# Autodesk Inventor assembly: zlozenie_ramka
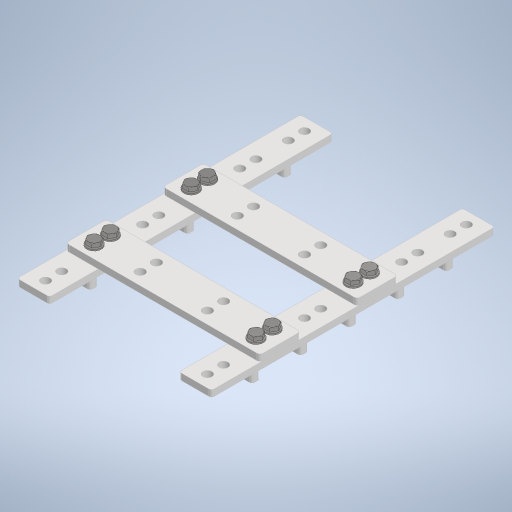
[picture p0: Inventor's stored thumbnail of the model, 512x512]
Saved by Autodesk Inventor 2024.2 (Build 282272000, 272)
## iProperties
Created: 2024-01-20
Part Number: zlozenie_ramka
Document SubType Name: Assembly
Designer: Konrad
Author: Konrad
## Documents named in this file (6)
- D:\Inventor\magisterka\prototyp_2\zlozenie_ramka.iam
- D:\Inventor\magisterka\prototyp_2\belka_poprzeg.ipt
- D:\Inventor\magisterka\prototyp_2\belka_wzdluz.ipt
- C:\Users\Konrad\Documents\Inventor\Content Center Files\R2024\pl-PL\DIN 125-1  A\DIN 125 - A 4,3.ipt
- C:\Users\Konrad\Documents\Inventor\Content Center Files\R2024\pl-PL\DIN EN 24 017\ISO 4017 - M4 x 16DIN EN.ipt
- C:\Users\Konrad\Documents\Inventor\Content Center Files\R2024\pl-PL\DIN 934\DIN 934 - M4 x 0,7.ipt
## Components (28 placed, 5 different names)
1. belka_poprzeg:1 — Zestawiające:1, Zestawiające:2, Równoległe:1, Równoległe:2, Zestawiające:4, Zestawiające:25, Zestawiające:27, Zestawiające:29, Zestawiające:31, Zestawiające:33, Zestawiające:35, Zestawiające:37, Zestawiające:39, Zestawiające:40, Zestawiające:41
2. belka_wzdluz:1 — Zestawiające:2, Równoległe:1, Zestawiające:4, Zestawiające:6, Zestawiające:16, Zestawiające:18, Zestawiające:20, Zestawiające:22, Zestawiające:32, Zestawiające:34, Zestawiające:36, Zestawiające:38
3. belka_poprzeg:2 — Zestawiające:3, Zestawiające:6, Zestawiające:42
4. belka_wzdluz:2 — Zestawiające:1, Równoległe:2, Zestawiające:3, Zestawiające:8, Zestawiające:9, Zestawiające:10, Zestawiające:11, Zestawiające:12, Zestawiające:13, Zestawiające:14, Zestawiające:15, Zestawiające:17, Zestawiające:19, Zestawiające:21, Zestawiające:23, Zestawiające:24, Zestawiające:26, Zestawiające:28, Zestawiające:30, Zestawiające:41, Zestawiające:42
5. DIN 125-1 A A 4,3:1 — Zestawiające:8, Zestawiające:9, Wstawiające:1
6. DIN EN 24017 M4 x 16:1 — Wstawiające:1
7. DIN 934 - zastąpiona przez DIN EN 24032/28673/28674 M4:1 — Zestawiające:24, Zestawiające:25
8. DIN 125-1 A A 4,3:2 — Zestawiające:10, Zestawiające:11, Wstawiające:2
9. DIN 125-1 A A 4,3:3 — Zestawiające:12, Zestawiające:13, Wstawiające:3
10. DIN 125-1 A A 4,3:4 — Zestawiające:14, Zestawiające:15, Wstawiające:4
11. DIN 125-1 A A 4,3:5 — Zestawiające:16, Zestawiające:17, Wstawiające:5
12. DIN 125-1 A A 4,3:6 — Zestawiające:18, Zestawiające:19, Wstawiające:6
13. DIN 125-1 A A 4,3:7 — Zestawiające:20, Zestawiające:21, Wstawiające:7
14. DIN 125-1 A A 4,3:8 — Zestawiające:22, Zestawiające:23, Wstawiające:8
15. DIN EN 24017 M4 x 16:2 — Wstawiające:2
16. DIN EN 24017 M4 x 16:3 — Wstawiające:3
17. DIN EN 24017 M4 x 16:4 — Wstawiające:4
18. DIN EN 24017 M4 x 16:5 — Wstawiające:5
19. DIN EN 24017 M4 x 16:6 — Wstawiające:6
20. DIN EN 24017 M4 x 16:7 — Wstawiające:7
21. DIN EN 24017 M4 x 16:8 — Wstawiające:8
22. DIN 934 - zastąpiona przez DIN EN 24032/28673/28674 M4:2 — Zestawiające:26, Zestawiające:27
23. DIN 934 - zastąpiona przez DIN EN 24032/28673/28674 M4:3 — Zestawiające:28, Zestawiające:29
24. DIN 934 - zastąpiona przez DIN EN 24032/28673/28674 M4:4 — Zestawiające:30, Zestawiające:31
25. DIN 934 - zastąpiona przez DIN EN 24032/28673/28674 M4:5 — Zestawiające:32, Zestawiające:33
26. DIN 934 - zastąpiona przez DIN EN 24032/28673/28674 M4:6 — Zestawiające:34, Zestawiające:35
27. DIN 934 - zastąpiona przez DIN EN 24032/28673/28674 M4:7 — Zestawiające:36, Zestawiające:37
28. DIN 934 - zastąpiona przez DIN EN 24032/28673/28674 M4:8 — Zestawiające:38, Zestawiające:39
## Relationships (50: Mate 40, Insert 8, Flush 2)
- Zestawiające:1 [Mate]: belka_poprzeg:1 ↔ belka_wzdluz:2
- Zestawiające:2 [Mate]: belka_poprzeg:1 ↔ belka_wzdluz:1
- Równoległe:1 [Flush]: belka_poprzeg:1 ↔ belka_wzdluz:1
- Równoległe:2 [Flush]: belka_poprzeg:1 ↔ belka_wzdluz:2
- Zestawiające:3 [Mate]: belka_poprzeg:2 ↔ belka_wzdluz:2
- Zestawiające:4 [Mate]: belka_poprzeg:1 ↔ belka_wzdluz:1
- Zestawiające:6 [Mate]: belka_wzdluz:1 ↔ belka_poprzeg:2
- Zestawiające:8 [Mate]: belka_wzdluz:2 ↔ DIN 125-1 A A 4,3:1
- Zestawiające:9 [Mate]: belka_wzdluz:2 ↔ DIN 125-1 A A 4,3:1
- Zestawiające:10 [Mate]: belka_wzdluz:2 ↔ DIN 125-1 A A 4,3:2
- Zestawiające:11 [Mate]: belka_wzdluz:2 ↔ DIN 125-1 A A 4,3:2
- Zestawiające:12 [Mate]: belka_wzdluz:2 ↔ DIN 125-1 A A 4,3:3
- Zestawiające:13 [Mate]: belka_wzdluz:2 ↔ DIN 125-1 A A 4,3:3
- Zestawiające:14 [Mate]: belka_wzdluz:2 ↔ DIN 125-1 A A 4,3:4
- Zestawiające:15 [Mate]: belka_wzdluz:2 ↔ DIN 125-1 A A 4,3:4
- Zestawiające:16 [Mate]: belka_wzdluz:1 ↔ DIN 125-1 A A 4,3:5
- Zestawiające:17 [Mate]: belka_wzdluz:2 ↔ DIN 125-1 A A 4,3:5
- Zestawiające:18 [Mate]: belka_wzdluz:1 ↔ DIN 125-1 A A 4,3:6
- Zestawiające:19 [Mate]: belka_wzdluz:2 ↔ DIN 125-1 A A 4,3:6
- Zestawiające:20 [Mate]: belka_wzdluz:1 ↔ DIN 125-1 A A 4,3:7
- Zestawiające:21 [Mate]: belka_wzdluz:2 ↔ DIN 125-1 A A 4,3:7
- Zestawiające:22 [Mate]: belka_wzdluz:1 ↔ DIN 125-1 A A 4,3:8
- Zestawiające:23 [Mate]: belka_wzdluz:2 ↔ DIN 125-1 A A 4,3:8
- Wstawiające:1 [Insert]: DIN 125-1 A A 4,3:1 ↔ DIN EN 24017 M4 x 16:1
- Wstawiające:2 [Insert]: DIN 125-1 A A 4,3:2 ↔ DIN EN 24017 M4 x 16:2
- Wstawiające:3 [Insert]: DIN 125-1 A A 4,3:3 ↔ DIN EN 24017 M4 x 16:3
- Wstawiające:4 [Insert]: DIN 125-1 A A 4,3:4 ↔ DIN EN 24017 M4 x 16:4
- Wstawiające:5 [Insert]: DIN 125-1 A A 4,3:5 ↔ DIN EN 24017 M4 x 16:5
- Wstawiające:6 [Insert]: DIN 125-1 A A 4,3:6 ↔ DIN EN 24017 M4 x 16:6
- Wstawiające:7 [Insert]: DIN 125-1 A A 4,3:7 ↔ DIN EN 24017 M4 x 16:7
- Wstawiające:8 [Insert]: DIN 125-1 A A 4,3:8 ↔ DIN EN 24017 M4 x 16:8
- Zestawiające:24 [Mate]: belka_wzdluz:2 ↔ DIN 934 - zastąpiona przez DIN EN 24032/28673/28674 M4:1
- Zestawiające:25 [Mate]: belka_poprzeg:1 ↔ DIN 934 - zastąpiona przez DIN EN 24032/28673/28674 M4:1
- Zestawiające:26 [Mate]: belka_wzdluz:2 ↔ DIN 934 - zastąpiona przez DIN EN 24032/28673/28674 M4:2
- Zestawiające:27 [Mate]: belka_poprzeg:1 ↔ DIN 934 - zastąpiona przez DIN EN 24032/28673/28674 M4:2
- Zestawiające:28 [Mate]: belka_wzdluz:2 ↔ DIN 934 - zastąpiona przez DIN EN 24032/28673/28674 M4:3
- Zestawiające:29 [Mate]: belka_poprzeg:1 ↔ DIN 934 - zastąpiona przez DIN EN 24032/28673/28674 M4:3
- Zestawiające:30 [Mate]: belka_wzdluz:2 ↔ DIN 934 - zastąpiona przez DIN EN 24032/28673/28674 M4:4
- Zestawiające:31 [Mate]: belka_poprzeg:1 ↔ DIN 934 - zastąpiona przez DIN EN 24032/28673/28674 M4:4
- Zestawiające:32 [Mate]: belka_wzdluz:1 ↔ DIN 934 - zastąpiona przez DIN EN 24032/28673/28674 M4:5
- Zestawiające:33 [Mate]: belka_poprzeg:1 ↔ DIN 934 - zastąpiona przez DIN EN 24032/28673/28674 M4:5
- Zestawiające:34 [Mate]: belka_wzdluz:1 ↔ DIN 934 - zastąpiona przez DIN EN 24032/28673/28674 M4:6
- Zestawiające:35 [Mate]: belka_poprzeg:1 ↔ DIN 934 - zastąpiona przez DIN EN 24032/28673/28674 M4:6
- Zestawiające:36 [Mate]: belka_wzdluz:1 ↔ DIN 934 - zastąpiona przez DIN EN 24032/28673/28674 M4:7
- Zestawiające:37 [Mate]: belka_poprzeg:1 ↔ DIN 934 - zastąpiona przez DIN EN 24032/28673/28674 M4:7
- Zestawiające:38 [Mate]: belka_wzdluz:1 ↔ DIN 934 - zastąpiona przez DIN EN 24032/28673/28674 M4:8
- Zestawiające:39 [Mate]: belka_poprzeg:1 ↔ DIN 934 - zastąpiona przez DIN EN 24032/28673/28674 M4:8
- Zestawiające:40 [Mate]: belka_poprzeg:1
- Zestawiające:41 [Mate]: belka_poprzeg:1 ↔ belka_wzdluz:2
- Zestawiające:42 [Mate]: belka_poprzeg:2 ↔ belka_wzdluz:2
